# Autodesk Inventor assembly: Pickup
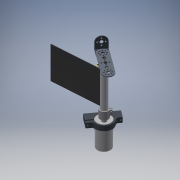
[picture p0: Inventor's stored thumbnail of the model, 180x180]
Saved by Autodesk Inventor 2016 (Build 200138000, 138)
## iProperties
Created: 2015-11-25
Part Number: Pickup
Document SubType Name: Assembly
Designer: Julia
Author: Julia
## Documents named in this file (10)
- C:\Users\Aeolus\Documents\GitHub\RobotuxCAD\Team Robotux 15-16 Robot Cad Assets\Pickup.iam
- C:\Users\Aeolus\Documents\GitHub\RobotuxCAD\Team Robotux 15-16 Robot Cad Assets\Pickup Pvc.ipt
- C:\Users\Aeolus\Documents\GitHub\RobotuxCAD\Team Robotux 15-16 Robot Cad Assets\tube_clamp_2012.ipt
- C:\Users\Aeolus\Documents\GitHub\RobotuxCAD\Team Robotux 15-16 Robot Cad Assets\Tetrix Parts\tetrix_739079_collar_2012.ipt
- C:\Users\Aeolus\Documents\GitHub\RobotuxCAD\Team Robotux 15-16 Robot Cad Assets\Pickup Flap.ipt
- C:\Users\Aeolus\Documents\GitHub\RobotuxCAD\Team Robotux 15-16 Robot Cad Assets\Tetrix Parts\tetrix_739172_2012.ipt
- C:\Users\Aeolus\Documents\GitHub\RobotuxCAD\Team Robotux 15-16 Robot Cad Assets\Tetrix Parts\tetrix_739062_2012.ipt
- C:\Users\Aeolus\Documents\GitHub\RobotuxCAD\Team Robotux 15-16 Robot Cad Assets\Tetrix Parts\tetrix_739273_2013.ipt
- C:\Users\Aeolus\Documents\GitHub\RobotuxCAD\Team Robotux 15-16 Robot Cad Assets\Tetrix Motor.ipt
- C:\Users\Aeolus\Documents\GitHub\RobotuxCAD\Team Robotux 15-16 Robot Cad Assets\Tetrix Parts\tetrix_739089_2012.ipt
## Components (10 placed, 9 different names)
1. Pickup Pvc:1 — Mate:6, Mate:7, Mate:8, Mate:17, Mate:18
2. tube_clamp_2012:1 — Mate:3, Mate:4, Mate:5, Mate:6, Flush:2
3. tube_clamp_2012:2 — Mate:8, Mate:9, Flush:2, Mate:10, Mate:11
4. tetrix_739079_collar_2012:1 — Mate:2, Mate:3, Mate:4, Mate:19
5. Pickup Flap:1 — Mate:17, Mate:18
6. tetrix_739172_2012:1 — Mate:10, Mate:11, Mate:12, Mate:13, Mate:20
7. tetrix_739062_2012:1 — Mate:14, Mate:15, Mate:16
8. tetrix_739273_2013:1 — Mate:13, Mate:14, Mate:15, Mate:16, Mate:20
9. Tetrix Motor:1 — Flush:1, Mate:1, Mate:2, Mate:5, Mate:7, Mate:9, Mate:12, Mate:19
10. tetrix_739089_2012:1 — Flush:1, Mate:1
## Relationships (22: Mate 20, Flush 2)
- Flush:1: Tetrix Motor:1 ↔ tetrix_739089_2012:1
- Mate:1: Tetrix Motor:1 ↔ tetrix_739089_2012:1
- Mate:2: tetrix_739079_collar_2012:1 ↔ Tetrix Motor:1
- Mate:3: tube_clamp_2012:1 ↔ tetrix_739079_collar_2012:1
- Mate:4: tube_clamp_2012:1 ↔ tetrix_739079_collar_2012:1
- Mate:5: tube_clamp_2012:1 ↔ Tetrix Motor:1
- Mate:6: Pickup Pvc:1 ↔ tube_clamp_2012:1
- Mate:7: Pickup Pvc:1 ↔ Tetrix Motor:1
- Mate:8: Pickup Pvc:1 ↔ tube_clamp_2012:2
- Mate:9: tube_clamp_2012:2 ↔ Tetrix Motor:1
- Flush:2: tube_clamp_2012:1 ↔ tube_clamp_2012:2
- Mate:10: tube_clamp_2012:2 ↔ tetrix_739172_2012:1
- Mate:11: tube_clamp_2012:2 ↔ tetrix_739172_2012:1
- Mate:12: tetrix_739172_2012:1 ↔ Tetrix Motor:1
- Mate:13: tetrix_739172_2012:1 ↔ tetrix_739273_2013:1
- Mate:14: tetrix_739062_2012:1 ↔ tetrix_739273_2013:1
- Mate:15: tetrix_739062_2012:1 ↔ tetrix_739273_2013:1
- Mate:16: tetrix_739062_2012:1 ↔ tetrix_739273_2013:1
- Mate:17: Pickup Pvc:1 ↔ Pickup Flap:1
- Mate:18: Pickup Pvc:1 ↔ Pickup Flap:1
- Mate:19: tetrix_739079_collar_2012:1 ↔ Tetrix Motor:1
- Mate:20: tetrix_739172_2012:1 ↔ tetrix_739273_2013:1
